# Autodesk Inventor assembly: (Unsaved)
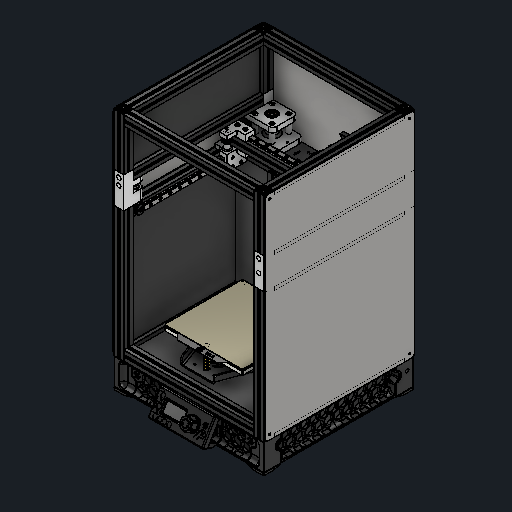
[picture p0: Inventor's stored thumbnail of the model, 512x512]
Saved by Autodesk Inventor 2026.1 (Build 301233020, 233B)
## iProperties
Created: 2025-05-09
Part Number: (Unsaved)
Document SubType Name: Assembly
Designer: AdminForWorker
Title: Voron 0 v2
Author: AdminForWorker
## Documents named in this file (19)
- C:\Users\JoshuaEah\Documents\GitHub\Voron-0\CAD\Voron 0.iam
- C:\Users\JoshuaEah\Documents\GitHub\Voron-0\CAD\Frame\Frame.iam
- C:\Users\JoshuaEah\Documents\GitHub\Voron-0\CAD\Skirt\Skirts.iam
- C:\Users\JoshuaEah\Documents\GitHub\Voron-0\CAD\Hardware\Electronics\Electronics.iam
- C:\Users\JoshuaEah\Documents\GitHub\Voron-0\CAD\Extras\Filament Spool.iam
- C:\Users\JoshuaEah\Documents\GitHub\Voron-0\CAD\Z Axis\Bed Assembly.iam
- C:\Users\JoshuaEah\Documents\GitHub\Voron-0\CAD\Z Axis\Z Motor Assembly.iam
- C:\Users\JoshuaEah\Documents\GitHub\Voron-0\CAD\Z Axis\Z Extrusion Right.iam
- Z Extrusion Right.iam
- C:\Users\JoshuaEah\Documents\GitHub\Voron-0\CAD\Z Axis\Z Extrusion Left.iam
- C:\Users\JoshuaEah\Documents\GitHub\Voron-0\CAD\Hardware\Linear Rail\Parts\MGN7H Carriage.ipt
- C:\Users\JoshuaEah\Documents\GitHub\Voron-0\CAD\Belts\Belts.iam
- C:\Users\JoshuaEah\Documents\GitHub\Voron-0\CAD\X Axis\X Axis.iam
- C:\Users\JoshuaEah\Documents\GitHub\Voron-0\CAD\Toolhead\Mini Stealthburner.iam
- C:\Users\JoshuaEah\Documents\GitHub\Voron-0\CAD\Enclosure\Enclosure.iam
- C:\Users\JoshuaEah\Documents\GitHub\Voron-0\CAD\Idlers\A Idler Assembly.iam
- C:\Users\JoshuaEah\Documents\GitHub\Voron-0\CAD\Idlers\B Idler Assembly.iam
- C:\Users\JoshuaEah\Documents\GitHub\Voron-0\CAD\AB Drives\A_Drive.iam
- C:\Users\JoshuaEah\Documents\GitHub\Voron-0\CAD\AB Drives\B_Drive.iam
## Components (21 placed, 21 different names)
1. Frame:1 [sub-assembly] — Flush:3, Angle:1, Mate:4, Cylindrical:5, Insert:7, Insert:8, Mate:22, Mate:23, Insert:9, Insert:10, Insert:11, Insert:12, Angle:3, Cylindrical:13, Angle:4
2. Belts:1 [sub-assembly]
3. A_Drive:1 [sub-assembly] — Insert:7, Mate:23
4. B_Drive:1 [sub-assembly] — Insert:8, Mate:22
5. A Idler Assembly:1 [sub-assembly] — Insert:9, Insert:10
6. B Idler Assembly:1 [sub-assembly] — Insert:11, Insert:12
7. X Axis:1 [sub-assembly] — Insert:13, Insert:14, Cylindrical:12, Angle:2
8. MGN7H X Carriage:1 — Cylindrical:12, Insert:15, Insert:16, Angle:2
9. Mini Stealthburner:1 [sub-assembly] — Insert:15, Insert:16
10. MGN7H Y Left Carriage:1 — Cylindrical:5, Insert:13, Angle:3
11. MGN7H Y Right Carriage:1 — Insert:14, Cylindrical:13, Angle:4
12. Bed Assembly:1 [sub-assembly] — Mate:1, Insert:1, Insert:2, Insert:3, Insert:4
13. Z Motor Assembly:1 [sub-assembly] — Mate:1, Flush:3, Angle:1
14. Z Extrusion Right:1 [sub-assembly] — Cylindrical:15, Angle:6
15. Z Extrusion Left:1 [sub-assembly] — Mate:4, Cylindrical:14, Angle:5
16. MGN7H Z Left Carriage:1 — Insert:2, Insert:3, Cylindrical:14, Angle:5
17. MGN7H Z Right Carriage:1 — Insert:1, Insert:4, Cylindrical:15, Angle:6
18. Skirts:1 [sub-assembly]
19. Enclosure:1 [sub-assembly]
20. Electronics:1 [sub-assembly]
21. Filament Spool:1 [sub-assembly]
## Relationships (52: Mate 17, Insert 14, Flush 10, Angle 6, CylindricalJoint 5)
- Mate:1: Bed Assembly:1 ↔ Z Motor Assembly:1
- [Mate]: Frame:1 ↔ Z Extrusion Right:1
- [Mate]: Frame:1 ↔ Z Extrusion Left:1
- [Flush]: Frame:1 ↔ Z Extrusion Right:1
- [Flush]: Frame:1 ↔ Z Extrusion Left:1
- Insert:1: Bed Assembly:1 ↔ MGN7H Z Right Carriage:1
- Insert:2: Bed Assembly:1 ↔ MGN7H Z Left Carriage:1
- Insert:3: Bed Assembly:1 ↔ MGN7H Z Left Carriage:1
- Insert:4: Bed Assembly:1 ↔ MGN7H Z Right Carriage:1
- Flush:3: Frame:1 ↔ Z Motor Assembly:1
- Angle:1 (0 deg): Frame:1 ↔ Z Motor Assembly:1
- Mate:4 (58 mm): Frame:1 ↔ Z Extrusion Left:1
- [Flush]: Bed Assembly:1 ↔ Z Extrusion Right:1
- Cylindrical:5: Frame:1 ↔ MGN7H Y Left Carriage:1
- [Mate]: Frame:1 ↔ Enclosure:1
- [Flush]: Frame:1 ↔ Enclosure:1
- [Flush]: Frame:1 ↔ Enclosure:1
- [Mate]: Frame:1 ↔ Enclosure:1
- [Flush]: Frame:1 ↔ Enclosure:1
- [Flush]: Frame:1 ↔ Enclosure:1
- [Mate]: Frame:1 ↔ Enclosure:1
- [Flush]: Frame:1 ↔ Enclosure:1
- [Flush]: Frame:1 ↔ Enclosure:1
- [Mate] (0.5 mm): Frame:1 ↔ Enclosure:1
- [Mate] (1 mm): Frame:1 ↔ Enclosure:1
- [Mate] (0.5 mm): Frame:1 ↔ Enclosure:1
- [Mate] (0.5 mm): Frame:1 ↔ Enclosure:1
- [Mate] (0.5 mm): Frame:1 ↔ Enclosure:1
- [Mate] (0.5 mm): Frame:1 ↔ Enclosure:1
- [Mate] (0.5 mm): Frame:1 ↔ Enclosure:1
- [Mate] (0.5 mm): Frame:1 ↔ Enclosure:1
- Insert:7: Frame:1 ↔ A_Drive:1
- Insert:8: Frame:1 ↔ B_Drive:1
- Mate:22: Frame:1 ↔ B_Drive:1
- Mate:23: Frame:1 ↔ A_Drive:1
- Insert:9: Frame:1 ↔ A Idler Assembly:1
- Insert:10: Frame:1 ↔ A Idler Assembly:1
- Insert:11: Frame:1 ↔ B Idler Assembly:1
- Insert:12: Frame:1 ↔ B Idler Assembly:1
- Insert:13: X Axis:1 ↔ MGN7H Y Left Carriage:1
- Insert:14: X Axis:1 ↔ MGN7H Y Right Carriage:1
- Cylindrical:12: X Axis:1 ↔ MGN7H X Carriage:1
- Insert:15: MGN7H X Carriage:1 ↔ Mini Stealthburner:1
- Insert:16: MGN7H X Carriage:1 ↔ Mini Stealthburner:1
- Angle:2 (0 deg): X Axis:1 ↔ MGN7H X Carriage:1
- Angle:3 (0 deg): Frame:1 ↔ MGN7H Y Left Carriage:1
- Cylindrical:13: Frame:1 ↔ MGN7H Y Right Carriage:1
- Angle:4 (0 deg): Frame:1 ↔ MGN7H Y Right Carriage:1
- Cylindrical:14: Z Extrusion Left:1 ↔ MGN7H Z Left Carriage:1
- Angle:5 (0 deg): Z Extrusion Left:1 ↔ MGN7H Z Left Carriage:1
- Cylindrical:15: Z Extrusion Right:1 ↔ MGN7H Z Right Carriage:1
- Angle:6 (0 deg): Z Extrusion Right:1 ↔ MGN7H Z Right Carriage:1
